# Autodesk Inventor assembly: ensambleLora32
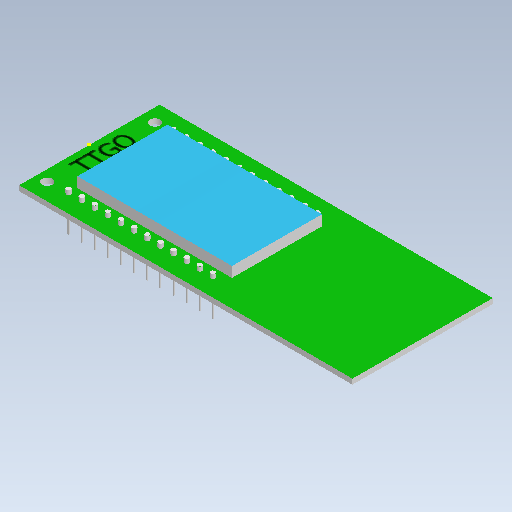
[picture p0: Inventor's stored thumbnail of the model, 512x512]
Saved by Autodesk Inventor 2020 (Build 240168000, 168)
## iProperties
Created: 2021-10-19
Part Number: ensambleLora32
Document SubType Name: Assembly
Designer: DANIEL
Author: DANIEL
## Documents named in this file (3)
- C:\Users\DANIEL\Documents\Personal\Convocatorias\Escollera\tesis\CAD\ensambleLora32.iam
- C:\Users\DANIEL\Documents\Personal\Convocatorias\Escollera\tesis\CAD\lora32Placa.ipt
- C:\Users\DANIEL\Documents\Personal\Convocatorias\Escollera\tesis\CAD\pata.ipt
## Components (25 placed, 2 different names)
1. lora32Placa:1 — Rígido:1, Rígido:2, Rígido:3, Rígido:4, Rígido:5, Rígido:6, Rígido:7, Rígido:8, Rígido:9, Rígido:10, Rígido:12, Rígido:13, Rígido:14, Rígido:15, Rígido:16, Rígido:17, Rígido:18, Rígido:19, Rígido:20, Rígido:21, Rígido:22, Rígido:23, Rígido:24, Rígido:25
2. pata:1 — Rígido:1
3. pata:2 — Rígido:2
4. pata:3 — Rígido:3
5. pata:4 — Rígido:4
6. pata:5 — Rígido:5
7. pata:6 — Rígido:6
8. pata:7 — Rígido:8
9. pata:8 — Rígido:16
10. pata:9 — Rígido:7
11. pata:10 — Rígido:9
12. pata:11 — Rígido:25
13. pata:12 — Rígido:10
14. pata:13 — Rígido:21
15. pata:14 — Rígido:22
16. pata:15 — Rígido:15
17. pata:16 — Rígido:13
18. pata:17 — Rígido:12
19. pata:18 — Rígido:14
20. pata:19 — Rígido:20
21. pata:20 — Rígido:24
22. pata:21 — Rígido:23
23. pata:22 — Rígido:19
24. pata:24 — Rígido:18
25. pata:26 — Rígido:17
## Relationships (24: WeldJoint 24)
- Rígido:1 [WeldJoint]: lora32Placa:1 ↔ pata:1
- Rígido:2 [WeldJoint]: lora32Placa:1 ↔ pata:2
- Rígido:3 [WeldJoint]: lora32Placa:1 ↔ pata:3
- Rígido:4 [WeldJoint]: lora32Placa:1 ↔ pata:4
- Rígido:5 [WeldJoint]: lora32Placa:1 ↔ pata:5
- Rígido:6 [WeldJoint]: lora32Placa:1 ↔ pata:6
- Rígido:7 [WeldJoint]: lora32Placa:1 ↔ pata:9
- Rígido:8 [WeldJoint]: lora32Placa:1 ↔ pata:7
- Rígido:9 [WeldJoint]: lora32Placa:1 ↔ pata:10
- Rígido:10 [WeldJoint]: lora32Placa:1 ↔ pata:12
- Rígido:12 [WeldJoint]: lora32Placa:1 ↔ pata:17
- Rígido:13 [WeldJoint]: lora32Placa:1 ↔ pata:16
- Rígido:14 [WeldJoint]: lora32Placa:1 ↔ pata:18
- Rígido:15 [WeldJoint]: lora32Placa:1 ↔ pata:15
- Rígido:16 [WeldJoint]: lora32Placa:1 ↔ pata:8
- Rígido:17 [WeldJoint]: lora32Placa:1 ↔ pata:26
- Rígido:18 [WeldJoint]: lora32Placa:1 ↔ pata:24
- Rígido:19 [WeldJoint]: lora32Placa:1 ↔ pata:22
- Rígido:20 [WeldJoint]: lora32Placa:1 ↔ pata:19
- Rígido:21 [WeldJoint]: lora32Placa:1 ↔ pata:13
- Rígido:22 [WeldJoint]: lora32Placa:1 ↔ pata:14
- Rígido:23 [WeldJoint]: lora32Placa:1 ↔ pata:21
- Rígido:24 [WeldJoint]: lora32Placa:1 ↔ pata:20
- Rígido:25 [WeldJoint]: lora32Placa:1 ↔ pata:11
